# Autodesk Inventor assembly: Haed
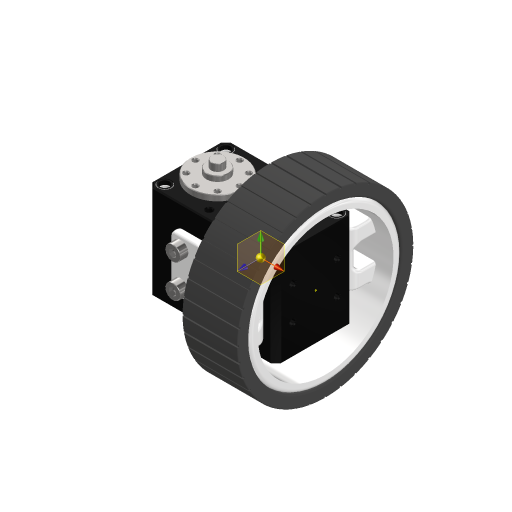
[picture p0: Inventor's stored thumbnail of the model, 512x512]
Saved by Autodesk Inventor 2024 (Build 280153000, 153)
## iProperties
Created: 2022-11-03
Part Number: Haed
Document SubType Name: Assembly
Designer: doore
Mass: 116.475 g
Surface Area: 323.603 cm^2
Volume: 75.9973 cm^3
Density: 1.53262 g/cm^3
Author: doore
## Documents named in this file (5)
- C:\Users\Bong\project\snake_RL\matlab\meshes\Inventor_Reallign\head\head.iam
- C:\Users\Bong\project\snake_RL\matlab\meshes\Inventor_Reallign\head\xm430.ipt
- C:\Users\Bong\project\snake_RL\matlab\meshes\Inventor_Reallign\head\solid_circular_frame.ipt
- C:\Users\Bong\Documents\Inventor\Content Center Files\R2024\ko-KR\BS EN ISO 4762\BS EN ISO 4762 - M3 x 5(1).ipt
- C:\Users\Bong\project\snake_RL\matlab\meshes\Inventor_Reallign\head\rubber.ipt
## Components (7 placed, 4 different names)
1. xm430:1 — 강체:1, 플러쉬:1, 메이트:1, 플러쉬:2
2. solid_circular_frame:1 — 강체:1, 강체:2, 강체:3, 강체:4, 강체:5, 강체:6
3. BS EN ISO 4762 : 부품 1 6각 소켓 머리 캡 나사 - 미터 M3 x 5:1 — 강체:2
4. BS EN ISO 4762 : 부품 1 6각 소켓 머리 캡 나사 - 미터 M3 x 5:2 — 강체:3
5. BS EN ISO 4762 : 부품 1 6각 소켓 머리 캡 나사 - 미터 M3 x 5:3 — 강체:4
6. BS EN ISO 4762 : 부품 1 6각 소켓 머리 캡 나사 - 미터 M3 x 5:4 — 강체:5
7. rubber:1 — 강체:6
## Relationships (9: WeldJoint 6, Flush 2, Mate 1)
- 강체:1 [WeldJoint]: xm430:1 ↔ solid_circular_frame:1
- 강체:2 [WeldJoint]: solid_circular_frame:1 ↔ BS EN ISO 4762 : 부품 1 6각 소켓 머리 캡 나사 - 미터 M3 x 5:1
- 강체:3 [WeldJoint]: solid_circular_frame:1 ↔ BS EN ISO 4762 : 부품 1 6각 소켓 머리 캡 나사 - 미터 M3 x 5:2
- 강체:4 [WeldJoint]: solid_circular_frame:1 ↔ BS EN ISO 4762 : 부품 1 6각 소켓 머리 캡 나사 - 미터 M3 x 5:3
- 강체:5 [WeldJoint]: solid_circular_frame:1 ↔ BS EN ISO 4762 : 부품 1 6각 소켓 머리 캡 나사 - 미터 M3 x 5:4
- 강체:6 [WeldJoint]: solid_circular_frame:1 ↔ rubber:1
- 플러쉬:1 [Flush]: xm430:1
- 메이트:1 [Mate]: xm430:1
- 플러쉬:2 [Flush]: xm430:1
